# Autodesk Inventor assembly: AS_Мехатрон R1
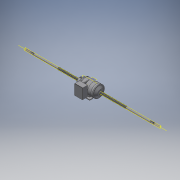
[picture p0: Inventor's stored thumbnail of the model, 180x180]
Saved by Autodesk Inventor 2016 SP1 (Build 200210100, 210)
## iProperties
Created: 2016-04-25
Part Number: AS_Мехатрон R1
Material: Типовые
Document SubType Name: Assembly
Designer: AS
Author: AS
## Documents named in this file (11)
- H:\Projects\GitHub\mechatron\AS_Мехатрон R1.iam
- H:\Projects\GitHub\mechatron\Vint.ipt
- H:\Projects\GitHub\mechatron\2 крышка.ipt
- H:\Projects\GitHub\mechatron\Деталь 3.ipt
- H:\Projects\GitHub\mechatron\Деталь 4.ipt
- H:\Projects\GitHub\mechatron\Деталь 5.ipt
- H:\Projects\GitHub\mechatron\Деталь 6.ipt
- H:\Projects\GitHub\mechatron\Полый вал.iam
- H:\Projects\GitHub\mechatron\Корпус 1 сборка.iam
- H:\Projects\GitHub\mechatron\AS_Мехатрон R1\Мастер проектирования\Болтовое соединение1.iam
- H:\Projects\GitHub\mechatron\AS_Мехатрон R1\Мастер проектирования\Болтовое соединение3.iam
## Components (18 placed, 9 different names)
1. Vint:1 — Совмещение:1
2. 2 крышка:1 — Заподлицо:2, Совмещение:3, Совмещение:11, Совмещение:15, Совмещение:19, Совмещение:20
3. Деталь 3:1 — Заподлицо:4, Совмещение:4, Совмещение:16, Совмещение:17
4. Деталь 4:1 — Заподлицо:5, Совмещение:5, Совмещение:7, Совмещение:17, Совмещение:18
5. Деталь 5:1 — Совмещение:6, Совмещение:11, Совмещение:12, Заподлицо:10, Совмещение:13, Совмещение:14
6. Деталь 6:1 — Заподлицо:7, Совмещение:7, Совмещение:18
7. Полый вал:1 [sub-assembly] — Совмещение:9, Совмещение:12, Заподлицо:10
8. Корпус 1 сборка:1 [sub-assembly] — Совмещение:10, Заподлицо:8, Заподлицо:9, Совмещение:15, Совмещение:16
9. Болтовое соединение:1 [sub-assembly] — Совмещение:13, Совмещение:14
10. Болтовое соединение:2 [sub-assembly]
11. Болтовое соединение:3 [sub-assembly]
12. Болтовое соединение:4 [sub-assembly]
13. Болтовое соединение:5 [sub-assembly] — Совмещение:19, Совмещение:20
14. Болтовое соединение:6 [sub-assembly]
15. Болтовое соединение:7 [sub-assembly]
16. Болтовое соединение:8 [sub-assembly]
17. Болтовое соединение:9 [sub-assembly]
18. Болтовое соединение:10 [sub-assembly]
## Component patterns: (4 elements, first: Болтовое соединение:1), (6 elements, first: Болтовое соединение:5)
## Relationships (25: Mate 18, Flush 7)
- Совмещение:1 [Mate]: Vint:1
- Заподлицо:2 [Flush]: 2 крышка:1
- Совмещение:3 [Mate]: 2 крышка:1
- Заподлицо:4 [Flush]: Деталь 3:1
- Совмещение:4 [Mate]: Деталь 3:1
- Заподлицо:5 [Flush]: Деталь 4:1
- Совмещение:5 [Mate]: Деталь 4:1
- Совмещение:6 [Mate]: Деталь 5:1
- Заподлицо:7 [Flush]: Деталь 6:1
- Совмещение:7 [Mate]: Деталь 4:1 ↔ Деталь 6:1
- Совмещение:9 [Mate]: Полый вал:1
- Совмещение:10 [Mate]: Корпус 1 сборка:1
- Заподлицо:8 [Flush]: Корпус 1 сборка:1
- Заподлицо:9 [Flush]: Корпус 1 сборка:1
- Совмещение:11 [Mate]: 2 крышка:1 ↔ Деталь 5:1
- Совмещение:12 [Mate]: Деталь 5:1 ↔ Полый вал:1
- Заподлицо:10 [Flush]: Деталь 5:1 ↔ Полый вал:1
- Совмещение:13 [Mate]: Деталь 5:1 ↔ Болтовое соединение:1
- Совмещение:14 [Mate]: Деталь 5:1 ↔ Болтовое соединение:1
- Совмещение:15 [Mate]: 2 крышка:1 ↔ Корпус 1 сборка:1
- Совмещение:16 [Mate]: Деталь 3:1 ↔ Корпус 1 сборка:1
- Совмещение:17 [Mate]: Деталь 3:1 ↔ Деталь 4:1
- Совмещение:18 [Mate]: Деталь 4:1 ↔ Деталь 6:1
- Совмещение:19 [Mate]: 2 крышка:1 ↔ Болтовое соединение:5
- Совмещение:20 [Mate]: 2 крышка:1 ↔ Болтовое соединение:5
